# Autodesk Inventor assembly: Ensamble_Conjunto
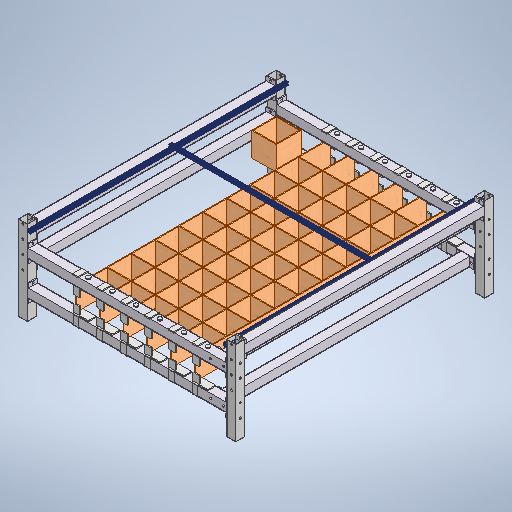
[picture p0: Inventor's stored thumbnail of the model, 512x512]
Saved by Autodesk Inventor 2025.2 (Build 292293000, 293)
## iProperties
Created: 2025-05-13
Part Number: Ensamble_Conjunto
Document SubType Name: Assembly
Designer: USER
Author: USER
## Documents named in this file (10)
- C:\Users\USER\Desktop\TESIS\STORAGE\Individual\Ensamble_Conjunto.iam
- C:\Users\USER\Desktop\TESIS\STORAGE\Subensamble estaciones.iam
- C:\Users\USER\Desktop\TESIS\STORAGE\Individual\Perfil_Vertical.ipt
- C:\Users\USER\Desktop\TESIS\STORAGE\Sujetadores.ipt
- C:\Users\USER\Desktop\TESIS\STORAGE\Sujetador2.ipt
- C:\Users\USER\Desktop\TESIS\STORAGE\Individual\Bases_perfiles.ipt
- C:\Users\USER\Desktop\TESIS\STORAGE\Individual\Bases_Fijas.ipt
- C:\Users\USER\Desktop\TESIS\STORAGE\Conjunto\Perfil_Horizontal.ipt
- C:\Users\USER\Desktop\TESIS\STORAGE\Conjunto\Perfil_Vertical20.ipt
- C:\Users\USER\Desktop\TESIS\STORAGE\Conjunto\Estacion.ipt
## Components (42 placed, 9 different names)
1. Subensamble estaciones:1 [sub-assembly] — Mate:3, Mate:4, Mate:5, Mate:15, Mate:16, Mate:19, Mate:22, Mate:25, Mate:38, Mate:39, Mate:40, Mate:41, Mate:42, Mate:43, Mate:44, Mate:45, Mate:70, Mate:71, Mate:72, Mate:73, Mate:74, Mate:75, Mate:76, Mate:77, Mate:78, Mate:91, Mate:92, Mate:93, Mate:94, Mate:95, Mate:96, Mate:97, Mate:98, Flush:8, Flush:9
2. Perfil_Vertical:1 — Mate:1, Mate:2, Mate:11, Mate:12, Mate:13, Mate:14, Mate:17, Mate:18, Mate:20, Mate:21, Mate:23, Mate:24, Mate:101, Mate:113
3. Sujetadores:1 — Mate:1, Mate:2, Mate:3, Mate:4, Mate:5
4. Sujetadores:2 — Mate:11, Mate:12, Mate:15
5. Sujetadores:3 — Mate:13, Mate:14, Mate:16
6. Sujetadores:4 — Mate:17, Mate:18, Mate:19
7. Sujetadores:5 — Mate:20, Mate:21, Mate:22
8. Sujetadores:6 — Mate:23, Mate:24, Mate:25
9. Perfil_Vertical:2 — Mate:26, Mate:27, Mate:28, Mate:29, Mate:30, Mate:31, Mate:32, Mate:33, Mate:34, Mate:35, Mate:36, Mate:37, Mate:102, Mate:110, Mate:111, Mate:112, Mate:117, Mate:118, Mate:119
10. Sujetador2:1 — Mate:26, Mate:27, Mate:38, Mate:39, Mate:40
11. Sujetador2:2 — Mate:28, Mate:29, Mate:41
12. Sujetador2:3 — Mate:30, Mate:31, Mate:42
13. Sujetador2:4 — Mate:36, Mate:37, Mate:45
14. Sujetador2:5 — Mate:32, Mate:33, Mate:43
15. Sujetador2:6 — Mate:34, Mate:35, Mate:44
16. Perfil_Vertical:4 — Mate:58, Mate:59, Mate:60, Mate:61, Mate:62, Mate:63, Mate:64, Mate:65, Mate:66, Mate:67, Mate:68, Mate:69, Mate:103, Mate:104, Mate:105, Mate:107, Mate:114
17. Sujetadores:7 — Mate:64, Mate:65, Mate:76
18. Sujetadores:8 — Mate:66, Mate:67, Mate:75, Mate:77
19. Sujetadores:9 — Mate:68, Mate:69, Mate:78
20. Sujetadores:10 — Mate:60, Mate:61, Mate:73
21. Sujetadores:11 — Mate:58, Mate:59, Mate:70, Mate:71, Mate:72
22. Sujetadores:12 — Mate:62, Mate:63, Mate:74
23. Perfil_Vertical:5 — Mate:79, Mate:80, Mate:81, Mate:82, Mate:83, Mate:84, Mate:85, Mate:86, Mate:87, Mate:88, Mate:89, Mate:90, Mate:99, Mate:100, Mate:106, Mate:108, Mate:109, Mate:115, Mate:116
24. Sujetador2:8 — Mate:85, Mate:86, Mate:96
25. Sujetador2:9 — Mate:79, Mate:80, Mate:91, Mate:92, Mate:93
26. Sujetador2:10 — Mate:87, Mate:88, Mate:97
27. Sujetador2:11 — Mate:83, Mate:84, Mate:95
28. Sujetador2:12 — Mate:89, Mate:90, Mate:98
29. Sujetador2:14 — Mate:81, Mate:82, Mate:94
30. Bases_perfiles:1 — Mate:102, Mate:103, Mate:104, Mate:105
31. Bases_perfiles:2 — Mate:99, Mate:100, Mate:101, Mate:106
32. Bases_Fijas:1 — Mate:107, Mate:108, Mate:109, Mate:126, Mate:127, Mate:130, Mate:131, Flush:5
33. Bases_Fijas:2 — Mate:110, Mate:111, Mate:112, Mate:113, Mate:128, Mate:129
34. Bases_Fijas:3 — Mate:114, Mate:115, Mate:116, Mate:120, Mate:121, Flush:2, Mate:134, Mate:135
35. Bases_Fijas:4 — Mate:117, Mate:118, Mate:119, Mate:122, Mate:123, Mate:124, Flush:1, Mate:136, Mate:137, Mate:138
36. Bases_perfiles:3 — Mate:120, Mate:121, Mate:122, Mate:123, Mate:124, Mate:125, Flush:3, Mate:141
37. Perfil_Horizontal:1 — Mate:125, Flush:1, Flush:2, Flush:3
38. Perfil_Horizontal:2 — Mate:132, Flush:4, Flush:5
39. Bases_perfiles:4 — Mate:126, Mate:127, Mate:128, Mate:129, Mate:130, Mate:131, Mate:132, Flush:4, Mate:133, Mate:140
40. Perfil_Vertical20:1 — Mate:133, Mate:140, Mate:141
41. Bases_perfiles:5 — Mate:134, Mate:135, Mate:136, Mate:137, Mate:138, Mate:139
42. Estacion:1 — Flush:8, Mate:139, Flush:9
## Relationships (131: Mate 124, Flush 7)
- Mate:1: Perfil_Vertical:1 ↔ Sujetadores:1
- Mate:2: Perfil_Vertical:1 ↔ Sujetadores:1
- Mate:3: Subensamble estaciones:1 ↔ Sujetadores:1
- Mate:4: Subensamble estaciones:1 ↔ Sujetadores:1
- Mate:5: Subensamble estaciones:1 ↔ Sujetadores:1
- Mate:11: Perfil_Vertical:1 ↔ Sujetadores:2
- Mate:12: Perfil_Vertical:1 ↔ Sujetadores:2
- Mate:13: Perfil_Vertical:1 ↔ Sujetadores:3
- Mate:14: Perfil_Vertical:1 ↔ Sujetadores:3
- Mate:15: Subensamble estaciones:1 ↔ Sujetadores:2
- Mate:16: Subensamble estaciones:1 ↔ Sujetadores:3
- Mate:17: Perfil_Vertical:1 ↔ Sujetadores:4
- Mate:18: Perfil_Vertical:1 ↔ Sujetadores:4
- Mate:19: Subensamble estaciones:1 ↔ Sujetadores:4
- Mate:20: Perfil_Vertical:1 ↔ Sujetadores:5
- Mate:21: Perfil_Vertical:1 ↔ Sujetadores:5
- Mate:22: Subensamble estaciones:1 ↔ Sujetadores:5
- Mate:23: Perfil_Vertical:1 ↔ Sujetadores:6
- Mate:24: Perfil_Vertical:1 ↔ Sujetadores:6
- Mate:25: Subensamble estaciones:1 ↔ Sujetadores:6
- Mate:26: Perfil_Vertical:2 ↔ Sujetador2:1
- Mate:27: Perfil_Vertical:2 ↔ Sujetador2:1
- Mate:28: Perfil_Vertical:2 ↔ Sujetador2:2
- Mate:29: Perfil_Vertical:2 ↔ Sujetador2:2
- Mate:30: Perfil_Vertical:2 ↔ Sujetador2:3
- Mate:31: Perfil_Vertical:2 ↔ Sujetador2:3
- Mate:32: Perfil_Vertical:2 ↔ Sujetador2:5
- Mate:33: Perfil_Vertical:2 ↔ Sujetador2:5
- Mate:34: Perfil_Vertical:2 ↔ Sujetador2:6
- Mate:35: Perfil_Vertical:2 ↔ Sujetador2:6
- Mate:36: Perfil_Vertical:2 ↔ Sujetador2:4
- Mate:37: Perfil_Vertical:2 ↔ Sujetador2:4
- Mate:38: Subensamble estaciones:1 ↔ Sujetador2:1
- Mate:39: Subensamble estaciones:1 ↔ Sujetador2:1
- Mate:40: Subensamble estaciones:1 ↔ Sujetador2:1
- Mate:41: Subensamble estaciones:1 ↔ Sujetador2:2
- Mate:42: Subensamble estaciones:1 ↔ Sujetador2:3
- Mate:43: Subensamble estaciones:1 ↔ Sujetador2:5
- Mate:44: Subensamble estaciones:1 ↔ Sujetador2:6
- Mate:45: Subensamble estaciones:1 ↔ Sujetador2:4
- Mate:58: Perfil_Vertical:4 ↔ Sujetadores:11
- Mate:59: Perfil_Vertical:4 ↔ Sujetadores:11
- Mate:60: Perfil_Vertical:4 ↔ Sujetadores:10
- Mate:61: Perfil_Vertical:4 ↔ Sujetadores:10
- Mate:62: Perfil_Vertical:4 ↔ Sujetadores:12
- Mate:63: Perfil_Vertical:4 ↔ Sujetadores:12
- Mate:64: Perfil_Vertical:4 ↔ Sujetadores:7
- Mate:65: Perfil_Vertical:4 ↔ Sujetadores:7
- Mate:66: Perfil_Vertical:4 ↔ Sujetadores:8
- Mate:67: Perfil_Vertical:4 ↔ Sujetadores:8
- Mate:68: Perfil_Vertical:4 ↔ Sujetadores:9
- Mate:69: Perfil_Vertical:4 ↔ Sujetadores:9
- Mate:70: Subensamble estaciones:1 ↔ Sujetadores:11
- Mate:71: Subensamble estaciones:1 ↔ Sujetadores:11
- Mate:72: Subensamble estaciones:1 ↔ Sujetadores:11
- Mate:73: Subensamble estaciones:1 ↔ Sujetadores:10
- Mate:74: Subensamble estaciones:1 ↔ Sujetadores:12
- Mate:75: Subensamble estaciones:1 ↔ Sujetadores:8
- Mate:76: Subensamble estaciones:1 ↔ Sujetadores:7
- Mate:77: Subensamble estaciones:1 ↔ Sujetadores:8
- Mate:78: Subensamble estaciones:1 ↔ Sujetadores:9
- Mate:79: Perfil_Vertical:5 ↔ Sujetador2:9
- Mate:80: Perfil_Vertical:5 ↔ Sujetador2:9
- Mate:81: Perfil_Vertical:5 ↔ Sujetador2:14
- Mate:82: Perfil_Vertical:5 ↔ Sujetador2:14
- Mate:83: Perfil_Vertical:5 ↔ Sujetador2:11
- Mate:84: Perfil_Vertical:5 ↔ Sujetador2:11
- Mate:85: Perfil_Vertical:5 ↔ Sujetador2:8
- Mate:86: Perfil_Vertical:5 ↔ Sujetador2:8
- Mate:87: Perfil_Vertical:5 ↔ Sujetador2:10
- Mate:88: Perfil_Vertical:5 ↔ Sujetador2:10
- Mate:89: Perfil_Vertical:5 ↔ Sujetador2:12
- Mate:90: Perfil_Vertical:5 ↔ Sujetador2:12
- Mate:91: Subensamble estaciones:1 ↔ Sujetador2:9
- Mate:92: Subensamble estaciones:1 ↔ Sujetador2:9
- Mate:93: Subensamble estaciones:1 ↔ Sujetador2:9
- Mate:94: Subensamble estaciones:1 ↔ Sujetador2:14
- Mate:95: Subensamble estaciones:1 ↔ Sujetador2:11
- Mate:96: Subensamble estaciones:1 ↔ Sujetador2:8
- Mate:97: Subensamble estaciones:1 ↔ Sujetador2:10
- Mate:98: Subensamble estaciones:1 ↔ Sujetador2:12
- Mate:99: Perfil_Vertical:5 ↔ Bases_perfiles:2
- Mate:100: Perfil_Vertical:5 ↔ Bases_perfiles:2
- Mate:101: Perfil_Vertical:1 ↔ Bases_perfiles:2
- Mate:102: Perfil_Vertical:2 ↔ Bases_perfiles:1
- Mate:103: Perfil_Vertical:4 ↔ Bases_perfiles:1
- Mate:104: Perfil_Vertical:4 ↔ Bases_perfiles:1
- Mate:105: Perfil_Vertical:4 ↔ Bases_perfiles:1
- Mate:106: Perfil_Vertical:5 ↔ Bases_perfiles:2
- Mate:107: Perfil_Vertical:4 ↔ Bases_Fijas:1
- Mate:108: Perfil_Vertical:5 ↔ Bases_Fijas:1
- Mate:109: Perfil_Vertical:5 ↔ Bases_Fijas:1
- Mate:110: Perfil_Vertical:2 ↔ Bases_Fijas:2
- Mate:111: Perfil_Vertical:2 ↔ Bases_Fijas:2
- Mate:112: Perfil_Vertical:2 ↔ Bases_Fijas:2
- Mate:113: Perfil_Vertical:1 ↔ Bases_Fijas:2
- Mate:114: Perfil_Vertical:4 ↔ Bases_Fijas:3
- Mate:115: Perfil_Vertical:5 ↔ Bases_Fijas:3
- Mate:116: Perfil_Vertical:5 ↔ Bases_Fijas:3
- Mate:117: Perfil_Vertical:2 ↔ Bases_Fijas:4
- Mate:118: Perfil_Vertical:2 ↔ Bases_Fijas:4
- Mate:119: Perfil_Vertical:2 ↔ Bases_Fijas:4
- Mate:120: Bases_Fijas:3 ↔ Bases_perfiles:3
- Mate:121: Bases_Fijas:3 ↔ Bases_perfiles:3
- Mate:122: Bases_Fijas:4 ↔ Bases_perfiles:3
- Mate:123: Bases_Fijas:4 ↔ Bases_perfiles:3
- Mate:124: Bases_Fijas:4 ↔ Bases_perfiles:3
- Mate:125: Bases_perfiles:3 ↔ Perfil_Horizontal:1
- Flush:1: Bases_Fijas:4 ↔ Perfil_Horizontal:1
- Flush:2: Bases_Fijas:3 ↔ Perfil_Horizontal:1
- Flush:3: Bases_perfiles:3 ↔ Perfil_Horizontal:1
- Mate:126: Bases_Fijas:1 ↔ Bases_perfiles:4
- Mate:127: Bases_Fijas:1 ↔ Bases_perfiles:4
- Mate:128: Bases_Fijas:2 ↔ Bases_perfiles:4
- Mate:129: Bases_Fijas:2 ↔ Bases_perfiles:4
- Mate:130: Bases_Fijas:1 ↔ Bases_perfiles:4
- Mate:131: Bases_Fijas:1 ↔ Bases_perfiles:4
- Mate:132: Perfil_Horizontal:2 ↔ Bases_perfiles:4
- Flush:4: Perfil_Horizontal:2 ↔ Bases_perfiles:4
- Flush:5: Bases_Fijas:1 ↔ Perfil_Horizontal:2
- Mate:133: Bases_perfiles:4 ↔ Perfil_Vertical20:1
- Mate:134: Bases_Fijas:3 ↔ Bases_perfiles:5
- Mate:135: Bases_Fijas:3 ↔ Bases_perfiles:5
- Mate:136: Bases_Fijas:4 ↔ Bases_perfiles:5
- Mate:137: Bases_Fijas:4 ↔ Bases_perfiles:5
- Mate:138: Bases_Fijas:4 ↔ Bases_perfiles:5
- Flush:8: Subensamble estaciones:1 ↔ Estacion:1
- Mate:139: Bases_perfiles:5 ↔ Estacion:1
- Mate:140: Bases_perfiles:4 ↔ Perfil_Vertical20:1
- Mate:141: Bases_perfiles:3 ↔ Perfil_Vertical20:1
- Flush:9: Subensamble estaciones:1 ↔ Estacion:1
